# Autodesk Inventor assembly: Millan Dart Assembly
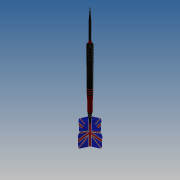
[picture p0: Inventor's stored thumbnail of the model, 180x180]
Saved by Autodesk Inventor 2018.2 (Build 222227000, 227)
## iProperties
Created: 2018-01-12
Part Number: Millan Dart Assembly
Document SubType Name: Assembly
Designer: Thomas Savage
Author: Thomas Savage
## Documents named in this file (3)
- G:\GrabCad\Millan Dart Assembly.iam
- G:\GrabCad\Millan Dart.ipt
- G:\GrabCad\Millan Dart Flight.ipt
## Components (3 placed, 2 different names)
1. Millan Dart:1
2. Millan Dart:2 — Mate:1
3. Millan Dart Flight:1 — Mate:1
## Relationships (1: Mate 1)
- Mate:1: Millan Dart:2 ↔ Millan Dart Flight:1
